# Autodesk Inventor assembly: palec
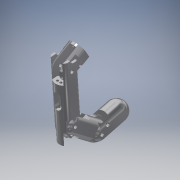
[picture p0: Inventor's stored thumbnail of the model, 180x180]
Saved by Autodesk Inventor 2019 (Build 230136000, 136)
## iProperties
Created: 2019-11-26
Part Number: palec
Document SubType Name: Assembly
Designer: Administrator
Title: Finger all pieces assembled v10
Author: Administrator
## Documents named in this file (6)
- C:\Users\wojta\Documents\Inventor\Reka\palec.iam
- C:\Users\wojta\Documents\Inventor\Reka\Base.ipt
- C:\Users\wojta\Documents\Inventor\Reka\Body.ipt
- C:\Users\wojta\Documents\Inventor\Reka\Middle.ipt
- C:\Users\wojta\Documents\Inventor\Reka\Tip.ipt
- C:\Users\wojta\Documents\Inventor\Reka\Lever korekta.ipt
## Components (5 placed, 5 different names)
1. Base:1 — Zestawiający:1, Zestawiający:2, Zestawiający:9, Zestawiający:10, Zestawiający:11
2. Body:1 — Zestawiający:1, Zestawiający:2
3. Middle:1 — Zestawiający:7, Zestawiający:8, Zestawiający:9, Zestawiający:10, Zestawiający:13
4. Tip:1 — Zestawiający:7, Zestawiający:8, Zestawiający:12
5. Lever korekta:1 — Zestawiający:11, Zestawiający:12, Zestawiający:13
## Relationships (9: Mate 9)
- Zestawiający:1 [Mate]: Base:1 ↔ Body:1
- Zestawiający:2 [Mate]: Base:1 ↔ Body:1
- Zestawiający:7 [Mate]: Middle:1 ↔ Tip:1
- Zestawiający:8 [Mate]: Middle:1 ↔ Tip:1
- Zestawiający:9 [Mate]: Base:1 ↔ Middle:1
- Zestawiający:10 [Mate]: Base:1 ↔ Middle:1
- Zestawiający:11 [Mate]: Base:1 ↔ Lever korekta:1
- Zestawiający:12 [Mate]: Tip:1 ↔ Lever korekta:1
- Zestawiający:13 [Mate]: Middle:1 ↔ Lever korekta:1
